# Autodesk Inventor assembly: Full payload assembly mk 2
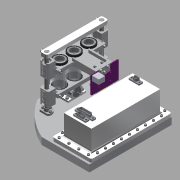
[picture p0: Inventor's stored thumbnail of the model, 180x180]
Saved by Autodesk Inventor 2017 (Build 210142000, 142)
## iProperties
Created: 2016-12-06
Part Number: Full payload assembly mk 2
Document SubType Name: Assembly
Designer: qupec
Mass: 896.86 g
Surface Area: 2165.29 cm^2
Volume: 326.413 cm^3
Density: 2.74763 g/cm^3
Author: qupec
## Documents named in this file (20)
- C:\Users\qupec\Desktop\UMD Near Space\STAR\CAD\Mechanical\Full payload assembly mk 2.iam
- C:\Users\qupec\Desktop\UMD Near Space\STAR\CAD\Mechanical\Slide rod assembly.iam
- C:\Users\qupec\Desktop\UMD Near Space\STAR\CAD\Mechanical\Test tube rack.iam
- C:\Users\qupec\Desktop\UMD Near Space\STAR\CAD\Mechanical\STARduino and Pi assembly.iam
- C:\Users\qupec\Desktop\UMD Near Space\STAR\CAD\Mechanical\Pi Cam and Cable assembly.iam
- C:\Users\qupec\Desktop\UMD Near Space\STAR\CAD\Mechanical\Ribbon Cable Connector-02.ipt
- C:\Users\qupec\Desktop\UMD Near Space\STAR\CAD\Mechanical\Full payload assembly\AIP\Cable and Harness\Full payload assembly.Harness2.iam
- C:\Users\qupec\Documents\Inventor\Content Center Files\R2017\en-US\U UNC 2603(1)\Unbrako - 4 x 1 - 48 - 1 - Unbrako.ipt
- C:\Users\qupec\Desktop\UMD Near Space\STAR\CAD\Mechanical\ShakerCAD\ShakerAssembly.iam
- C:\Users\qupec\Desktop\UMD Near Space\STAR\CAD\Mechanical\Base Plate Mk 2.ipt
- C:\Users\qupec\Desktop\UMD Near Space\STAR\CAD\Mechanical\Electronics Box.ipt
- C:\Users\qupec\Desktop\UMD Near Space\STAR\CAD\Mechanical\Sensor Board.ipt
- C:\Users\qupec\Desktop\UMD Near Space\STAR\CAD\Mechanical\9pin female connector.ipt
- C:\Users\qupec\Desktop\UMD Near Space\STAR\CAD\Mechanical\9pin male connector.ipt
- C:\Users\qupec\Desktop\UMD Near Space\STAR\CAD\Mechanical\31pin female connector.ipt
- C:\Users\qupec\Desktop\UMD Near Space\STAR\CAD\Mechanical\15pin female connector.ipt
- C:\Users\qupec\Documents\Inventor\Content Center Files\R2017\en-US\ANSI B18.3(05)\ANSI B18.3 - 3-48 UNC - 0.75(31).ipt
- C:\Users\qupec\Documents\Inventor\Content Center Files\R2017\en-US\ANSI B18.3(05)\ANSI B18.3 - 4-40 UNC - 0.625(31).ipt
- C:\Users\qupec\Documents\Inventor\Content Center Files\R2017\en-US\ANSI B18.3(05)\ANSI B18.3 - 4-40 UNC - 0.5(31).ipt
- C:\Users\qupec\Desktop\UMD Near Space\STAR\CAD\Mechanical\LED 5mm.ipt
## Components (56 placed, 19 different names)
1. Slide rod assembly:1 [sub-assembly] — Mate:119, Mate:120, Mate:121, Mate:278, Mate:280, Mate:282, Mate:284, Mate:286, Mate:288, Mate:290, Mate:292, Mate:294, Mate:296
2. Test tube rack:1 [sub-assembly] — Mate:56, Flush:19, Flush:20, Mate:113, Mate:114, Mate:119, Mate:120, Tangent:1
3. Pi Cam and Cable assembly:1 [sub-assembly] — Mate:56, Flush:19, Flush:20, Mate:161, Mate:162, Mate:169, Mate:171, Insert:1, Mate:299, Mate:300, Mate:302
4. Ribbon Cable Connector-02:1 — Mate:80, Flush:24, Flush:25
5. Harness2 [sub-assembly]
6. STARduino and Pi assembly:1 [sub-assembly] — Mate:80, Flush:24, Flush:25, Mate:122, Flush:41, Flush:42
7. ShakerAssembly:1 [sub-assembly] — Mate:113, Mate:114, Flush:26, Mate:123
8. Base Plate Mk 2:1 — Mate:121, Flush:26, Mate:122, Mate:123, Mate:124, Flush:29, Tangent:1, Flush:32, Mate:163, Flush:33, Flush:40, Mate:277, Mate:279, Mate:281, Mate:283, Mate:285, Mate:287, Mate:289, Mate:291, Mate:293, Mate:295
9. Sensor Board:1 — Mate:161, Mate:162, Angle:1, Mate:297, Mate:298
10. 9pin male connector:1
11. 31pin female connector:1 — Flush:34, Flush:35, Mate:164
12. 15pin female connector:1 — Mate:165, Flush:43, Flush:44
13. 9pin female connector:1 — Flush:38, Flush:39, Mate:166
14. Electronics Box:1 — Mate:163, Flush:33, Flush:34, Flush:35, Mate:164, Flush:38, Flush:39, Mate:165, Mate:166, Flush:40, Flush:41, Flush:42, Flush:43, Flush:44, Mate:225, Mate:226, Mate:227, Mate:228, Mate:229, Mate:230, Mate:231, Mate:232, Mate:233, Mate:234, Mate:235, Mate:236, Mate:237, Mate:238, Mate:239, Mate:240, Mate:241, Mate:242, Mate:243, Mate:244, Mate:245, Mate:246, Mate:247, Mate:248, Mate:249, Mate:250, Mate:251, Mate:252, Mate:253, Mate:254, Mate:255, Mate:256, Mate:257, Mate:258, Mate:259, Mate:260, Mate:261, Mate:262, Mate:263, Mate:264, Mate:265, Mate:266, Mate:267, Mate:268, Mate:269, Mate:270, Mate:271, Mate:272, Mate:273, Mate:274, Mate:275, Mate:276
15. Hexagon Socket Head Cap Screw - Inch No. 4 - 40 UNC - 1/2:1
16. Hexagon Socket Head Cap Screw - Inch No. 4 - 40 UNC - 1/2:2
17. Unbrako UNC Hex Socket Cap - Inch 4 x 1 - Unbrako:13 — Mate:169, Mate:171
18. Hexagon Socket Head Cap Screw - Inch No. 3 - 48 UNC - 3/4:2 — Mate:225, Mate:226
19. Hexagon Socket Head Cap Screw - Inch No. 3 - 48 UNC - 3/4:3 — Mate:227, Mate:228
20. Hexagon Socket Head Cap Screw - Inch No. 3 - 48 UNC - 3/4:4 — Mate:229, Mate:230
21. Hexagon Socket Head Cap Screw - Inch No. 3 - 48 UNC - 3/4:5 — Mate:231, Mate:232
22. Hexagon Socket Head Cap Screw - Inch No. 3 - 48 UNC - 3/4:6 — Mate:233, Mate:234
23. Hexagon Socket Head Cap Screw - Inch No. 3 - 48 UNC - 3/4:7 — Mate:235, Mate:236
24. Hexagon Socket Head Cap Screw - Inch No. 3 - 48 UNC - 3/4:8 — Mate:237, Mate:238
25. Hexagon Socket Head Cap Screw - Inch No. 3 - 48 UNC - 3/4:9 — Mate:239, Mate:240
26. Hexagon Socket Head Cap Screw - Inch No. 3 - 48 UNC - 3/4:10 — Mate:241, Mate:242
27. Hexagon Socket Head Cap Screw - Inch No. 3 - 48 UNC - 3/4:11 — Mate:243, Mate:244
28. Hexagon Socket Head Cap Screw - Inch No. 3 - 48 UNC - 3/4:12 — Mate:245, Mate:246
29. Hexagon Socket Head Cap Screw - Inch No. 3 - 48 UNC - 3/4:13 — Mate:247, Mate:248
30. Hexagon Socket Head Cap Screw - Inch No. 3 - 48 UNC - 3/4:14 — Mate:249, Mate:250
31. Hexagon Socket Head Cap Screw - Inch No. 3 - 48 UNC - 3/4:15 — Mate:251, Mate:252
32. Hexagon Socket Head Cap Screw - Inch No. 3 - 48 UNC - 3/4:16 — Mate:253, Mate:254
33. Hexagon Socket Head Cap Screw - Inch No. 3 - 48 UNC - 3/4:17 — Mate:255, Mate:256
34. Hexagon Socket Head Cap Screw - Inch No. 3 - 48 UNC - 3/4:18 — Mate:257, Mate:258
35. Hexagon Socket Head Cap Screw - Inch No. 3 - 48 UNC - 3/4:19 — Mate:259, Mate:260
36. Hexagon Socket Head Cap Screw - Inch No. 3 - 48 UNC - 3/4:20 — Mate:261, Mate:262
37. Hexagon Socket Head Cap Screw - Inch No. 3 - 48 UNC - 3/4:21 — Mate:263, Mate:264
38. Hexagon Socket Head Cap Screw - Inch No. 3 - 48 UNC - 3/4:22 — Mate:265, Mate:266
39. Hexagon Socket Head Cap Screw - Inch No. 3 - 48 UNC - 3/4:23 — Mate:267, Mate:268
40. Hexagon Socket Head Cap Screw - Inch No. 3 - 48 UNC - 3/4:24 — Mate:269, Mate:270
41. Hexagon Socket Head Cap Screw - Inch No. 3 - 48 UNC - 3/4:25 — Mate:271, Mate:272
42. Hexagon Socket Head Cap Screw - Inch No. 3 - 48 UNC - 3/4:26 — Mate:273, Mate:274
43. Hexagon Socket Head Cap Screw - Inch No. 3 - 48 UNC - 3/4:27 — Mate:275, Mate:276
44. Hexagon Socket Head Cap Screw - Inch No. 4 - 40 UNC - 5/8:1 — Mate:277, Mate:278
45. Hexagon Socket Head Cap Screw - Inch No. 4 - 40 UNC - 5/8:2 — Mate:279, Mate:280
46. Hexagon Socket Head Cap Screw - Inch No. 4 - 40 UNC - 5/8:3 — Mate:281, Mate:282
47. Hexagon Socket Head Cap Screw - Inch No. 4 - 40 UNC - 5/8:4 — Mate:283, Mate:284
48. Hexagon Socket Head Cap Screw - Inch No. 4 - 40 UNC - 5/8:5 — Mate:285, Mate:286
49. Hexagon Socket Head Cap Screw - Inch No. 4 - 40 UNC - 5/8:6 — Mate:287, Mate:288
50. Hexagon Socket Head Cap Screw - Inch No. 4 - 40 UNC - 5/8:7 — Mate:289, Mate:290
51. Hexagon Socket Head Cap Screw - Inch No. 4 - 40 UNC - 5/8:8 — Mate:291, Mate:292
52. Hexagon Socket Head Cap Screw - Inch No. 4 - 40 UNC - 5/8:9 — Mate:293, Mate:294
53. Hexagon Socket Head Cap Screw - Inch No. 4 - 40 UNC - 5/8:10 — Mate:295, Mate:296
54. Hexagon Socket Head Cap Screw - Inch No. 4 - 40 UNC - 5/8:11 — Insert:1
55. LED 5mm:1 — Mate:298, Mate:299, Mate:301, Mate:302
56. LED 5mm:2 — Mate:297, Mate:300, Mate:301
## Relationships (120: Mate 100, Flush 17, Tangent 1, Angle 1, Insert 1)
- Mate:56: Test tube rack:1 ↔ Pi Cam and Cable assembly:1
- Flush:19: Test tube rack:1 ↔ Pi Cam and Cable assembly:1
- Flush:20: Test tube rack:1 ↔ Pi Cam and Cable assembly:1
- Mate:80: Ribbon Cable Connector-02:1 ↔ STARduino and Pi assembly:1
- Flush:24 (-7 mm): Ribbon Cable Connector-02:1 ↔ STARduino and Pi assembly:1
- Flush:25: Ribbon Cable Connector-02:1 ↔ STARduino and Pi assembly:1
- Mate:113: Test tube rack:1 ↔ ShakerAssembly:1
- Mate:114: Test tube rack:1 ↔ ShakerAssembly:1
- Mate:119: Slide rod assembly:1 ↔ Test tube rack:1
- Mate:120: Slide rod assembly:1 ↔ Test tube rack:1
- Mate:121: Slide rod assembly:1 ↔ Base Plate Mk 2:1
- Flush:26 (5.08 mm): ShakerAssembly:1 ↔ Base Plate Mk 2:1
- Mate:122: STARduino and Pi assembly:1 ↔ Base Plate Mk 2:1
- Mate:123: ShakerAssembly:1 ↔ Base Plate Mk 2:1
- Mate:124: Base Plate Mk 2:1
- Flush:29: Base Plate Mk 2:1
- Tangent:1: Test tube rack:1 ↔ Base Plate Mk 2:1
- Mate:161: Pi Cam and Cable assembly:1 ↔ Sensor Board:1
- Mate:162: Pi Cam and Cable assembly:1 ↔ Sensor Board:1
- Flush:32: Base Plate Mk 2:1
- Angle:1 (0 deg): Sensor Board:1
- Mate:163: Base Plate Mk 2:1 ↔ Electronics Box:1
- Flush:33: Base Plate Mk 2:1 ↔ Electronics Box:1
- Flush:34 (12.7 mm): 31pin female connector:1 ↔ Electronics Box:1
- Flush:35 (6.35 mm): 31pin female connector:1 ↔ Electronics Box:1
- Mate:164: 31pin female connector:1 ↔ Electronics Box:1
- Flush:38 (6.35 mm): 9pin female connector:1 ↔ Electronics Box:1
- Flush:39 (-6.35 mm): 9pin female connector:1 ↔ Electronics Box:1
- Mate:165: 15pin female connector:1 ↔ Electronics Box:1
- Mate:166: 9pin female connector:1 ↔ Electronics Box:1
- Flush:40: Base Plate Mk 2:1 ↔ Electronics Box:1
- Flush:41: STARduino and Pi assembly:1 ↔ Electronics Box:1
- Flush:42: STARduino and Pi assembly:1 ↔ Electronics Box:1
- Flush:43 (3.81 mm): 15pin female connector:1 ↔ Electronics Box:1
- Flush:44 (12.7 mm): 15pin female connector:1 ↔ Electronics Box:1
- [Mate]: Pi Cam and Cable assembly:1 ↔ Hexagon Socket Head Cap Screw - Inch No. 4 - 40 UNC - 1/2:1
- [Mate]: Pi Cam and Cable assembly:1 ↔ Hexagon Socket Head Cap Screw - Inch No. 4 - 40 UNC - 1/2:2
- Mate:169: Pi Cam and Cable assembly:1 ↔ Unbrako UNC Hex Socket Cap - Inch 4 x 1 - Unbrako:13
- [Mate]: Pi Cam and Cable assembly:1 ↔ Hexagon Socket Head Cap Screw - Inch No. 4 - 40 UNC - 1/2:2
- Mate:171: Pi Cam and Cable assembly:1 ↔ Unbrako UNC Hex Socket Cap - Inch 4 x 1 - Unbrako:13
- [Mate]: Pi Cam and Cable assembly:1 ↔ Hexagon Socket Head Cap Screw - Inch No. 4 - 40 UNC - 1/2:1
- Mate:225: Electronics Box:1 ↔ Hexagon Socket Head Cap Screw - Inch No. 3 - 48 UNC - 3/4:2
- Mate:226: Electronics Box:1 ↔ Hexagon Socket Head Cap Screw - Inch No. 3 - 48 UNC - 3/4:2
- Mate:227: Electronics Box:1 ↔ Hexagon Socket Head Cap Screw - Inch No. 3 - 48 UNC - 3/4:3
- Mate:228: Electronics Box:1 ↔ Hexagon Socket Head Cap Screw - Inch No. 3 - 48 UNC - 3/4:3
- Mate:229: Electronics Box:1 ↔ Hexagon Socket Head Cap Screw - Inch No. 3 - 48 UNC - 3/4:4
- Mate:230: Electronics Box:1 ↔ Hexagon Socket Head Cap Screw - Inch No. 3 - 48 UNC - 3/4:4
- Mate:231: Electronics Box:1 ↔ Hexagon Socket Head Cap Screw - Inch No. 3 - 48 UNC - 3/4:5
- Mate:232: Electronics Box:1 ↔ Hexagon Socket Head Cap Screw - Inch No. 3 - 48 UNC - 3/4:5
- Mate:233: Electronics Box:1 ↔ Hexagon Socket Head Cap Screw - Inch No. 3 - 48 UNC - 3/4:6
- Mate:234: Electronics Box:1 ↔ Hexagon Socket Head Cap Screw - Inch No. 3 - 48 UNC - 3/4:6
- Mate:235: Electronics Box:1 ↔ Hexagon Socket Head Cap Screw - Inch No. 3 - 48 UNC - 3/4:7
- Mate:236: Electronics Box:1 ↔ Hexagon Socket Head Cap Screw - Inch No. 3 - 48 UNC - 3/4:7
- Mate:237: Electronics Box:1 ↔ Hexagon Socket Head Cap Screw - Inch No. 3 - 48 UNC - 3/4:8
- Mate:238: Electronics Box:1 ↔ Hexagon Socket Head Cap Screw - Inch No. 3 - 48 UNC - 3/4:8
- Mate:239: Electronics Box:1 ↔ Hexagon Socket Head Cap Screw - Inch No. 3 - 48 UNC - 3/4:9
- Mate:240: Electronics Box:1 ↔ Hexagon Socket Head Cap Screw - Inch No. 3 - 48 UNC - 3/4:9
- Mate:241: Electronics Box:1 ↔ Hexagon Socket Head Cap Screw - Inch No. 3 - 48 UNC - 3/4:10
- Mate:242: Electronics Box:1 ↔ Hexagon Socket Head Cap Screw - Inch No. 3 - 48 UNC - 3/4:10
- Mate:243: Electronics Box:1 ↔ Hexagon Socket Head Cap Screw - Inch No. 3 - 48 UNC - 3/4:11
- Mate:244: Electronics Box:1 ↔ Hexagon Socket Head Cap Screw - Inch No. 3 - 48 UNC - 3/4:11
- Mate:245: Electronics Box:1 ↔ Hexagon Socket Head Cap Screw - Inch No. 3 - 48 UNC - 3/4:12
- Mate:246: Electronics Box:1 ↔ Hexagon Socket Head Cap Screw - Inch No. 3 - 48 UNC - 3/4:12
- Mate:247: Electronics Box:1 ↔ Hexagon Socket Head Cap Screw - Inch No. 3 - 48 UNC - 3/4:13
- Mate:248: Electronics Box:1 ↔ Hexagon Socket Head Cap Screw - Inch No. 3 - 48 UNC - 3/4:13
- Mate:249: Electronics Box:1 ↔ Hexagon Socket Head Cap Screw - Inch No. 3 - 48 UNC - 3/4:14
- Mate:250: Electronics Box:1 ↔ Hexagon Socket Head Cap Screw - Inch No. 3 - 48 UNC - 3/4:14
- Mate:251: Electronics Box:1 ↔ Hexagon Socket Head Cap Screw - Inch No. 3 - 48 UNC - 3/4:15
- Mate:252: Electronics Box:1 ↔ Hexagon Socket Head Cap Screw - Inch No. 3 - 48 UNC - 3/4:15
- Mate:253: Electronics Box:1 ↔ Hexagon Socket Head Cap Screw - Inch No. 3 - 48 UNC - 3/4:16
- Mate:254: Electronics Box:1 ↔ Hexagon Socket Head Cap Screw - Inch No. 3 - 48 UNC - 3/4:16
- Mate:255: Electronics Box:1 ↔ Hexagon Socket Head Cap Screw - Inch No. 3 - 48 UNC - 3/4:17
- Mate:256: Electronics Box:1 ↔ Hexagon Socket Head Cap Screw - Inch No. 3 - 48 UNC - 3/4:17
- Mate:257: Electronics Box:1 ↔ Hexagon Socket Head Cap Screw - Inch No. 3 - 48 UNC - 3/4:18
- Mate:258: Electronics Box:1 ↔ Hexagon Socket Head Cap Screw - Inch No. 3 - 48 UNC - 3/4:18
- Mate:259: Electronics Box:1 ↔ Hexagon Socket Head Cap Screw - Inch No. 3 - 48 UNC - 3/4:19
- Mate:260: Electronics Box:1 ↔ Hexagon Socket Head Cap Screw - Inch No. 3 - 48 UNC - 3/4:19
- Mate:261: Electronics Box:1 ↔ Hexagon Socket Head Cap Screw - Inch No. 3 - 48 UNC - 3/4:20
- Mate:262: Electronics Box:1 ↔ Hexagon Socket Head Cap Screw - Inch No. 3 - 48 UNC - 3/4:20
- Mate:263: Electronics Box:1 ↔ Hexagon Socket Head Cap Screw - Inch No. 3 - 48 UNC - 3/4:21
- Mate:264: Electronics Box:1 ↔ Hexagon Socket Head Cap Screw - Inch No. 3 - 48 UNC - 3/4:21
- Mate:265: Electronics Box:1 ↔ Hexagon Socket Head Cap Screw - Inch No. 3 - 48 UNC - 3/4:22
- Mate:266: Electronics Box:1 ↔ Hexagon Socket Head Cap Screw - Inch No. 3 - 48 UNC - 3/4:22
- Mate:267: Electronics Box:1 ↔ Hexagon Socket Head Cap Screw - Inch No. 3 - 48 UNC - 3/4:23
- Mate:268: Electronics Box:1 ↔ Hexagon Socket Head Cap Screw - Inch No. 3 - 48 UNC - 3/4:23
- Mate:269: Electronics Box:1 ↔ Hexagon Socket Head Cap Screw - Inch No. 3 - 48 UNC - 3/4:24
- Mate:270: Electronics Box:1 ↔ Hexagon Socket Head Cap Screw - Inch No. 3 - 48 UNC - 3/4:24
- Mate:271: Electronics Box:1 ↔ Hexagon Socket Head Cap Screw - Inch No. 3 - 48 UNC - 3/4:25
- Mate:272: Electronics Box:1 ↔ Hexagon Socket Head Cap Screw - Inch No. 3 - 48 UNC - 3/4:25
- Mate:273: Electronics Box:1 ↔ Hexagon Socket Head Cap Screw - Inch No. 3 - 48 UNC - 3/4:26
- Mate:274: Electronics Box:1 ↔ Hexagon Socket Head Cap Screw - Inch No. 3 - 48 UNC - 3/4:26
- Mate:275: Electronics Box:1 ↔ Hexagon Socket Head Cap Screw - Inch No. 3 - 48 UNC - 3/4:27
- Mate:276: Electronics Box:1 ↔ Hexagon Socket Head Cap Screw - Inch No. 3 - 48 UNC - 3/4:27
- Mate:277: Base Plate Mk 2:1 ↔ Hexagon Socket Head Cap Screw - Inch No. 4 - 40 UNC - 5/8:1
- Mate:278: Slide rod assembly:1 ↔ Hexagon Socket Head Cap Screw - Inch No. 4 - 40 UNC - 5/8:1
- Mate:279: Base Plate Mk 2:1 ↔ Hexagon Socket Head Cap Screw - Inch No. 4 - 40 UNC - 5/8:2
- Mate:280: Slide rod assembly:1 ↔ Hexagon Socket Head Cap Screw - Inch No. 4 - 40 UNC - 5/8:2
- Mate:281: Base Plate Mk 2:1 ↔ Hexagon Socket Head Cap Screw - Inch No. 4 - 40 UNC - 5/8:3
- Mate:282: Slide rod assembly:1 ↔ Hexagon Socket Head Cap Screw - Inch No. 4 - 40 UNC - 5/8:3
- Mate:283: Base Plate Mk 2:1 ↔ Hexagon Socket Head Cap Screw - Inch No. 4 - 40 UNC - 5/8:4
- Mate:284: Slide rod assembly:1 ↔ Hexagon Socket Head Cap Screw - Inch No. 4 - 40 UNC - 5/8:4
- Mate:285: Base Plate Mk 2:1 ↔ Hexagon Socket Head Cap Screw - Inch No. 4 - 40 UNC - 5/8:5
- Mate:286: Slide rod assembly:1 ↔ Hexagon Socket Head Cap Screw - Inch No. 4 - 40 UNC - 5/8:5
- Mate:287: Base Plate Mk 2:1 ↔ Hexagon Socket Head Cap Screw - Inch No. 4 - 40 UNC - 5/8:6
- Mate:288: Slide rod assembly:1 ↔ Hexagon Socket Head Cap Screw - Inch No. 4 - 40 UNC - 5/8:6
- Mate:289: Base Plate Mk 2:1 ↔ Hexagon Socket Head Cap Screw - Inch No. 4 - 40 UNC - 5/8:7
- Mate:290: Slide rod assembly:1 ↔ Hexagon Socket Head Cap Screw - Inch No. 4 - 40 UNC - 5/8:7
- Mate:291: Base Plate Mk 2:1 ↔ Hexagon Socket Head Cap Screw - Inch No. 4 - 40 UNC - 5/8:8
- Mate:292: Slide rod assembly:1 ↔ Hexagon Socket Head Cap Screw - Inch No. 4 - 40 UNC - 5/8:8
- Mate:293: Base Plate Mk 2:1 ↔ Hexagon Socket Head Cap Screw - Inch No. 4 - 40 UNC - 5/8:9
- Mate:294: Slide rod assembly:1 ↔ Hexagon Socket Head Cap Screw - Inch No. 4 - 40 UNC - 5/8:9
- Mate:295: Base Plate Mk 2:1 ↔ Hexagon Socket Head Cap Screw - Inch No. 4 - 40 UNC - 5/8:10
- Mate:296: Slide rod assembly:1 ↔ Hexagon Socket Head Cap Screw - Inch No. 4 - 40 UNC - 5/8:10
- Insert:1: Pi Cam and Cable assembly:1 ↔ Hexagon Socket Head Cap Screw - Inch No. 4 - 40 UNC - 5/8:11
- Mate:297: Sensor Board:1 ↔ LED 5mm:2
- Mate:298: Sensor Board:1 ↔ LED 5mm:1
- Mate:299: Pi Cam and Cable assembly:1 ↔ LED 5mm:1
- Mate:300: Pi Cam and Cable assembly:1 ↔ LED 5mm:2
- Mate:301: LED 5mm:1 ↔ LED 5mm:2
- Mate:302: Pi Cam and Cable assembly:1 ↔ LED 5mm:1
